# Autodesk Inventor assembly: ASY MSC 080 gills
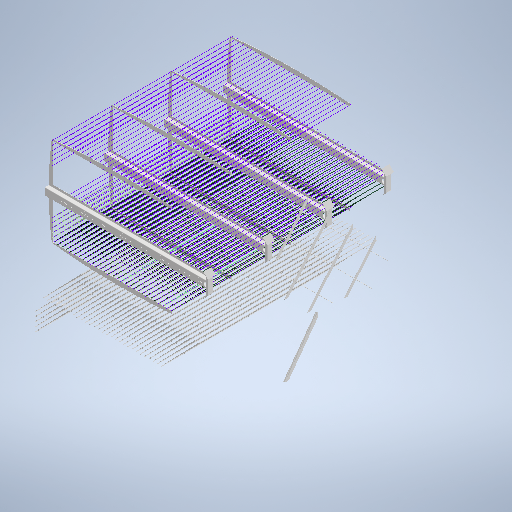
[picture p0: Inventor's stored thumbnail of the model, 512x512]
Saved by Autodesk Inventor 2025 (Build 290162010, 162A)
## iProperties
Created: 2024-08-31
Part Number: ASY MSC 080 gills
Document SubType Name: Assembly
Designer: pokla
Stock Number: ASY МОО 080 Жабры
Author: pokla
## Documents named in this file (25)
- C:\Users\DELL\YandexDisk-badmisterfox\домашниий пк\Inventor\Manturovo\Manturovo_Se-clar\ASY MSC 080 gills.iam
- C:\Users\DELL\YandexDisk-badmisterfox\домашниий пк\Inventor\Manturovo\Manturovo_Se-clar\MSC 802 sheet gills.ipt
- C:\Users\DELL\YandexDisk-badmisterfox\домашниий пк\Inventor\Manturovo\Manturovo_Se-clar\MSC 081 pillar gills.ipt
- C:\Users\DELL\YandexDisk-badmisterfox\домашниий пк\Inventor\Manturovo\Manturovo_Se-clar\MSC 804 sheet gills.ipt
- C:\Users\DELL\YandexDisk-badmisterfox\домашниий пк\Inventor\Manturovo\Manturovo_Se-clar\MSC 803 sheet gills.ipt
- C:\Users\DELL\YandexDisk-badmisterfox\домашниий пк\Inventor\Manturovo\Manturovo_Se-clar\MSC 806 sheet gills.ipt
- C:\Users\DELL\YandexDisk-badmisterfox\домашниий пк\Inventor\Manturovo\Manturovo_Se-clar\MSC 805 sheet gills.ipt
- C:\Users\DELL\YandexDisk-badmisterfox\домашниий пк\Inventor\Manturovo\Manturovo_Se-clar\MSC 808 sheet gills.ipt
- C:\Users\DELL\YandexDisk-badmisterfox\домашниий пк\Inventor\Manturovo\Manturovo_Se-clar\MSC 807 sheet gills.ipt
- C:\Users\DELL\YandexDisk-badmisterfox\домашниий пк\Inventor\Manturovo\Manturovo_Se-clar\MSC 810 sheet gills.ipt
- C:\Users\DELL\YandexDisk-badmisterfox\домашниий пк\Inventor\Manturovo\Manturovo_Se-clar\MSC 809 sheet gills.ipt
- C:\Users\DELL\YandexDisk-badmisterfox\домашниий пк\Inventor\Manturovo\Manturovo_Se-clar\MSC 812 sheet gills.ipt
- C:\Users\DELL\YandexDisk-badmisterfox\домашниий пк\Inventor\Manturovo\Manturovo_Se-clar\MSC 811 sheet gills.ipt
- C:\Users\DELL\YandexDisk-badmisterfox\домашниий пк\Inventor\Manturovo\Manturovo_Se-clar\MSC 084 wall support gills.ipt
- C:\Users\DELL\YandexDisk-badmisterfox\домашниий пк\Inventor\Manturovo\Manturovo_Se-clar\MSC 082 pillar gills.ipt
- C:\Users\DELL\YandexDisk-badmisterfox\домашниий пк\Inventor\Manturovo\Manturovo_Se-clar\MSC 086 string for sheets gills.ipt
- C:\Users\DELL\YandexDisk-badmisterfox\домашниий пк\Inventor\Manturovo\Manturovo_Se-clar\MSC 083 top support gills.ipt
- C:\Users\DELL\YandexDisk-badmisterfox\домашниий пк\Inventor\Manturovo\Manturovo_Se-clar\MSC 801 sheet gills.ipt
- C:\Users\DELL\YandexDisk-badmisterfox\домашниий пк\Inventor\Manturovo\Manturovo_Se-clar\ASY MSC 089 gills base.iam
- C:\Users\DELL\YandexDisk-badmisterfox\домашниий пк\Inventor\Manturovo\Manturovo_Se-clar\MSC 082 pillar 2.ipt
- C:\Users\DELL\YandexDisk-badmisterfox\домашниий пк\Inventor\Manturovo\Manturovo_Se-clar\MSC 0691 stringer cone.ipt
- C:\Users\DELL\YandexDisk-badmisterfox\домашниий пк\Inventor\Manturovo\Manturovo_Se-clar\конус\MSC 0161 stringer cone exit back.ipt
- C:\Users\DELL\YandexDisk-badmisterfox\домашниий пк\Inventor\Manturovo\Manturovo_Se-clar\конус\MSC 0162 stringer cone exit back.ipt
- C:\Users\DELL\YandexDisk-badmisterfox\домашниий пк\Inventor\Manturovo\Manturovo_Se-clar\конус\MSC 0163 rib cone exit back.ipt
- C:\Users\DELL\YandexDisk-badmisterfox\домашниий пк\Inventor\Manturovo\Manturovo_Se-clar\конус\MSC 0164 rib cone exit back.ipt
## Components (347 placed, 35 different names)
1. MSC 804 sheet gills:1 — Rigid:39
2. MSC 803 sheet gills:1 — Angle:2, Tangent:8, Tangent:9, Flush:15, Flush:19, Rigid:39
3. MSC 806 sheet gills:1 — Rigid:36
4. MSC 805 sheet gills:1 — Rigid:36, Angle:3, Tangent:10, Tangent:11, Flush:15, Flush:16
5. MSC 808 sheet gills:1 — Rigid:37
6. MSC 807 sheet gills:1 — Rigid:37, Angle:4, Tangent:12, Tangent:13, Flush:16, Flush:17
7. MSC 810 sheet gills:1 — Rigid:38
8. MSC 809 sheet gills:1 — Rigid:38, Angle:5, Tangent:17, Tangent:18, Flush:17, Flush:18
9. MSC 812 sheet gills:1 — Rigid:32
10. MSC 811 sheet gills:1 — Rigid:32, Angle:6, Tangent:19, Tangent:20, Flush:18
11. MSC 084 wall support gills:1 — Rigid:12, Rigid:25, Rigid:30, Tangent:14, Tangent:15
12. MSC 084 wall support gills:2 — Rigid:25, Rigid:26, Mate:17
13. MSC 084 wall support gills:3 — Rigid:26, Rigid:27
14. MSC 084 wall support gills:4 — Rigid:27
15. MSC 0103 sheet gills:2
16. MSC 0203 sheet gills:2
17. MSC 0104 sheet gills:2
18. MSC 0204 sheet gills:2
19. MSC 0105 sheet gills:2
20. MSC 0205 sheet gills:2
21. MSC 0106 sheet gills:2
22. MSC 0206 sheet gills:2
23. MSC 0107 sheet gills:2
24. MSC 0207 sheet gills:2
25. MSC 0161 stringer cone exit back:1
26. MSC 0162 stringer cone exit back:1
27. MSC 0161 stringer cone exit back:2
28. MSC 0162 stringer cone exit back:2
29. MSC 0163 rib cone exit back:1
30. MSC 0164 rib cone exit back:1
31. MSC 0163 rib cone exit back:2
32. MSC 081 pillar gills:1 — Rotational:1, Rotational:2, Tangent:16, Mate:18
33. MSC 082 pillar gills:1 — Rigid:28, Rigid:29
34. ASY MSC 089 gills base:1 [sub-assembly]
35. MSC 083 top support gills:1 — Rigid:24, Rigid:29, Rigid:31
36. MSC 083 top support gills:2 — Rigid:28, Rigid:30, Tangent:8, Tangent:9, Tangent:10, Tangent:11, Tangent:12, Tangent:13, Tangent:17, Tangent:18, Tangent:19, Tangent:20, Rigid:40
37. MSC 084 wall support gills:5 — Rigid:15, Rigid:31
38. MSC 081 pillar gills:2
39. MSC 082 pillar gills:2
40. ASY MSC 089 gills base:2 [sub-assembly]
41. MSC 083 top support gills:3
42. MSC 083 top support gills:6
43. MSC 084 wall support gills:6
44. MSC 081 pillar gills:3
45. MSC 082 pillar gills:3
46. ASY MSC 089 gills base:3 [sub-assembly]
47. MSC 083 top support gills:4
48. MSC 083 top support gills:7
49. MSC 084 wall support gills:7
50. MSC 081 pillar gills:4
51. MSC 082 pillar gills:4
52. ASY MSC 089 gills base:4 [sub-assembly]
53. MSC 083 top support gills:5
54. MSC 083 top support gills:8
55. MSC 084 wall support gills:8
56. MSC 801 sheet gills:1 — Mate:17, Rigid:33, Angle:2, Angle:3, Angle:4, Angle:5, Angle:6, Tangent:14, Tangent:15, Tangent:16, Flush:19
57. MSC 802 sheet gills:1 — Rigid:33
58. MSC 802 sheet gills:2
59. MSC 0201 sheet gills:2
60. MSC 0201 sheet gills:3
61. MSC 802 sheet gills:3
62. MSC 802 sheet gills:4
63. MSC 0201 sheet gills:4
64. MSC 0201 sheet gills:5
65. MSC 802 sheet gills:5
66. MSC 802 sheet gills:6
67. MSC 0201 sheet gills:6
68. MSC 0201 sheet gills:7
69. MSC 802 sheet gills:7
70. MSC 802 sheet gills:8
71. MSC 0201 sheet gills:8
72. MSC 0201 sheet gills:9
73. MSC 802 sheet gills:9
74. MSC 802 sheet gills:10
75. MSC 0201 sheet gills:10
76. MSC 0201 sheet gills:11
77. MSC 802 sheet gills:11
78. MSC 802 sheet gills:12
79. MSC 0201 sheet gills:12
80. MSC 0201 sheet gills:13
81. MSC 802 sheet gills:13
82. MSC 802 sheet gills:14
83. MSC 0201 sheet gills:14
84. MSC 0201 sheet gills:15
85. MSC 802 sheet gills:15
86. MSC 802 sheet gills:16
87. MSC 0201 sheet gills:16
88. MSC 0201 sheet gills:17
89. MSC 802 sheet gills:17
90. MSC 802 sheet gills:18
91. MSC 0201 sheet gills:18
92. MSC 0201 sheet gills:19
93. MSC 802 sheet gills:19
94. MSC 802 sheet gills:20
95. MSC 0201 sheet gills:20
96. MSC 0201 sheet gills:21
97. MSC 802 sheet gills:21
98. MSC 802 sheet gills:22
99. MSC 0201 sheet gills:22
100. MSC 0201 sheet gills:23
101. MSC 802 sheet gills:23
102. MSC 802 sheet gills:24
103. MSC 0201 sheet gills:24
104. MSC 0201 sheet gills:25
105. MSC 802 sheet gills:25
106. MSC 802 sheet gills:26
107. MSC 0201 sheet gills:26
108. MSC 0201 sheet gills:27
109. MSC 802 sheet gills:27
110. MSC 802 sheet gills:28
111. MSC 0201 sheet gills:28
112. MSC 0201 sheet gills:29
113. MSC 802 sheet gills:29
114. MSC 802 sheet gills:30
115. MSC 0201 sheet gills:30
116. MSC 0201 sheet gills:31
117. MSC 802 sheet gills:31
118. MSC 802 sheet gills:32
119. MSC 0201 sheet gills:32
120. MSC 0201 sheet gills:33
121. MSC 802 sheet gills:33
122. MSC 802 sheet gills:34
123. MSC 0201 sheet gills:34
124. MSC 0201 sheet gills:35
125. MSC 802 sheet gills:35
126. MSC 802 sheet gills:36
127. MSC 0201 sheet gills:36
128. MSC 0201 sheet gills:37
129. MSC 802 sheet gills:37
130. MSC 802 sheet gills:38
131. MSC 0201 sheet gills:38
132. MSC 0201 sheet gills:39
133. MSC 802 sheet gills:39
134. MSC 802 sheet gills:40
135. MSC 0201 sheet gills:40
136. MSC 0201 sheet gills:41
137. MSC 802 sheet gills:41
138. MSC 802 sheet gills:42
139. MSC 0201 sheet gills:42
140. MSC 0201 sheet gills:43
141. MSC 802 sheet gills:43
142. MSC 802 sheet gills:44
143. MSC 0201 sheet gills:44
144. MSC 0201 sheet gills:45
145. MSC 802 sheet gills:45
146. MSC 802 sheet gills:46
147. MSC 0201 sheet gills:46
148. MSC 0201 sheet gills:47
149. MSC 802 sheet gills:47
150. MSC 802 sheet gills:48
151. MSC 0201 sheet gills:48
152. MSC 0201 sheet gills:49
153. MSC 802 sheet gills:49
154. MSC 802 sheet gills:50
155. MSC 0201 sheet gills:50
156. MSC 0201 sheet gills:51
157. MSC 802 sheet gills:51
158. MSC 802 sheet gills:52
159. MSC 0201 sheet gills:52
160. MSC 0201 sheet gills:53
161. MSC 802 sheet gills:53
162. MSC 802 sheet gills:54
163. MSC 0201 sheet gills:54
164. MSC 0201 sheet gills:55
165. MSC 802 sheet gills:55
166. MSC 802 sheet gills:56
167. MSC 0201 sheet gills:56
168. MSC 0201 sheet gills:57
169. MSC 802 sheet gills:57
170. MSC 802 sheet gills:58
171. MSC 0201 sheet gills:58
172. MSC 086 string for sheets gills:1 — Rigid:12
173. MSC 086 string for sheets gills:2 — Rigid:15
174. MSC 086 string for sheets gills:3
175. MSC 086 string for sheets gills:344
176. MSC 086 string for sheets gills:5
177. MSC 086 string for sheets gills:345
178. MSC 086 string for sheets gills:7
179. MSC 086 string for sheets gills:346
180. MSC 086 string for sheets gills:9
181. MSC 086 string for sheets gills:347
182. MSC 086 string for sheets gills:11
183. MSC 086 string for sheets gills:348
184. MSC 086 string for sheets gills:13
185. MSC 086 string for sheets gills:349
186. MSC 086 string for sheets gills:15
187. MSC 086 string for sheets gills:350
188. MSC 086 string for sheets gills:17
189. MSC 086 string for sheets gills:351
190. MSC 086 string for sheets gills:19
191. MSC 086 string for sheets gills:352
192. MSC 086 string for sheets gills:21
193. MSC 086 string for sheets gills:353
194. MSC 086 string for sheets gills:23
195. MSC 086 string for sheets gills:354
196. MSC 086 string for sheets gills:25
197. MSC 086 string for sheets gills:355
198. MSC 086 string for sheets gills:27
199. MSC 086 string for sheets gills:356
200. MSC 086 string for sheets gills:29
201. MSC 086 string for sheets gills:357
202. MSC 086 string for sheets gills:31
203. MSC 086 string for sheets gills:358
204. MSC 086 string for sheets gills:33
205. MSC 086 string for sheets gills:359
206. MSC 086 string for sheets gills:35
207. MSC 086 string for sheets gills:360
208. MSC 086 string for sheets gills:37
209. MSC 086 string for sheets gills:361
210. MSC 086 string for sheets gills:39
211. MSC 086 string for sheets gills:362
212. MSC 086 string for sheets gills:41
213. MSC 086 string for sheets gills:363
214. MSC 086 string for sheets gills:43
215. MSC 086 string for sheets gills:364
216. MSC 086 string for sheets gills:45
217. MSC 086 string for sheets gills:365
218. MSC 086 string for sheets gills:47
219. MSC 086 string for sheets gills:366
220. MSC 086 string for sheets gills:49
221. MSC 086 string for sheets gills:367
222. MSC 086 string for sheets gills:51
223. MSC 086 string for sheets gills:368
224. MSC 086 string for sheets gills:53
225. MSC 086 string for sheets gills:369
226. MSC 086 string for sheets gills:55
227. MSC 086 string for sheets gills:370
228. MSC 086 string for sheets gills:58 — Rotational:1
229. MSC 086 string for sheets gills:57 — Rotational:2
230. MSC 082 pillar 2:1 — Mate:18
231. MSC 086 string for sheets gills:278
232. MSC 086 string for sheets gills:279
233. MSC 082 pillar 2:2
234. MSC 086 string for sheets gills:280
235. MSC 086 string for sheets gills:281
236. MSC 082 pillar 2:3
237. MSC 086 string for sheets gills:282
238. MSC 086 string for sheets gills:283
239. MSC 082 pillar 2:4
240. MSC 086 string for sheets gills:284
241. MSC 086 string for sheets gills:285
242. MSC 082 pillar 2:5
243. MSC 086 string for sheets gills:286
244. MSC 086 string for sheets gills:287
245. MSC 082 pillar 2:6
246. MSC 086 string for sheets gills:288
247. MSC 086 string for sheets gills:289
248. MSC 082 pillar 2:7
249. MSC 086 string for sheets gills:290
250. MSC 086 string for sheets gills:291
251. MSC 082 pillar 2:8
252. MSC 086 string for sheets gills:292
253. MSC 086 string for sheets gills:293
254. MSC 082 pillar 2:9
255. MSC 086 string for sheets gills:294
256. MSC 086 string for sheets gills:295
257. MSC 082 pillar 2:10
258. MSC 086 string for sheets gills:296
259. MSC 086 string for sheets gills:297
260. MSC 082 pillar 2:11
261. MSC 086 string for sheets gills:298
262. MSC 086 string for sheets gills:299
263. MSC 082 pillar 2:12
264. MSC 086 string for sheets gills:300
265. MSC 086 string for sheets gills:301
266. MSC 082 pillar 2:13
267. MSC 086 string for sheets gills:302
268. MSC 086 string for sheets gills:303
269. MSC 082 pillar 2:14
270. MSC 086 string for sheets gills:304
271. MSC 086 string for sheets gills:305
272. MSC 082 pillar 2:15
273. MSC 086 string for sheets gills:306
274. MSC 086 string for sheets gills:307
275. MSC 082 pillar 2:16
276. MSC 086 string for sheets gills:308
277. MSC 086 string for sheets gills:309
278. MSC 082 pillar 2:17
279. MSC 086 string for sheets gills:310
280. MSC 086 string for sheets gills:311
281. MSC 082 pillar 2:18
282. MSC 086 string for sheets gills:312
283. MSC 086 string for sheets gills:313
284. MSC 082 pillar 2:19
285. MSC 086 string for sheets gills:314
286. MSC 086 string for sheets gills:315
287. MSC 082 pillar 2:20
288. MSC 086 string for sheets gills:316
289. MSC 086 string for sheets gills:317
290. MSC 082 pillar 2:21
291. MSC 086 string for sheets gills:318
292. MSC 086 string for sheets gills:319
293. MSC 082 pillar 2:22
294. MSC 086 string for sheets gills:320
295. MSC 086 string for sheets gills:321
296. MSC 082 pillar 2:23
297. MSC 086 string for sheets gills:322
298. MSC 086 string for sheets gills:323
299. MSC 082 pillar 2:24
300. MSC 086 string for sheets gills:324
301. MSC 086 string for sheets gills:325
302. MSC 082 pillar 2:25
303. MSC 086 string for sheets gills:326
304. MSC 086 string for sheets gills:327
305. MSC 082 pillar 2:26
306. MSC 086 string for sheets gills:328
307. MSC 086 string for sheets gills:329
308. MSC 082 pillar 2:27
309. MSC 086 string for sheets gills:330
310. MSC 086 string for sheets gills:331
311. MSC 082 pillar 2:28
312. MSC 086 string for sheets gills:332
313. MSC 086 string for sheets gills:333
314. MSC 082 pillar 2:29
315. MSC 086 string for sheets gills:334
316. MSC 086 string for sheets gills:335
317. MSC 082 pillar 2:30
318. MSC 086 string for sheets gills:336
319. MSC 086 string for sheets gills:337
320. MSC 082 pillar 2:31
321. MSC 086 string for sheets gills:338
322. MSC 086 string for sheets gills:339
323. MSC 082 pillar 2:32
324. MSC 086 string for sheets gills:340
325. MSC 086 string for sheets gills:341
326. MSC 082 pillar 2:33
327. MSC 086 string for sheets gills:342
328. MSC 086 string for sheets gills:343
329. MSC 082 pillar 2:34
330. MSC 086 string for sheets gills:125 — Rigid:40
331. MSC 086 string for sheets gills:126
332. MSC 086 string for sheets gills:127
333. MSC 086 string for sheets gills:128
334. MSC 086 string for sheets gills:129
335. MSC 086 string for sheets gills:130
336. MSC 086 string for sheets gills:131 — Rigid:24
337. MSC 086 string for sheets gills:371
338. MSC 086 string for sheets gills:372
339. MSC 086 string for sheets gills:373
340. MSC 086 string for sheets gills:374
341. MSC 086 string for sheets gills:375
342. MSC 0691 stringer cone:1
343. MSC 0691 stringer cone:2
344. MSC 0691 stringer cone:3
345. MSC 0691 stringer cone:4
346. MSC 0691 stringer cone:5
347. MSC 0691 stringer cone:6
## Component patterns: (4 elements, first: MSC 081 pillar gills:1 + MSC 082 pillar gills:1 + ASY MSC 089 gills base:1 + MSC 083 top support gills:1 + MSC 083 top support gills:2 + MSC 084 wall support gills:5), (29 elements, first: MSC 801 sheet gills:1 + MSC 802 sheet gills:1 + MSC 802 sheet gills:2 + MSC 0201 sheet gills:2), (28 elements, first: MSC 086 string for sheets gills:1 + MSC 086 string for sheets gills:2), (34 elements, first: MSC 086 string for sheets gills:58 + MSC 086 string for sheets gills:57 + MSC 082 pillar 2:1), (6 elements, first: MSC 086 string for sheets gills:125), (6 elements, first: MSC 086 string for sheets gills:131), (6 elements, first: MSC 0691 stringer cone:1)
## Relationships (67: WeldJoint 30, Tangent 13, Flush 12, Mate 5, Angle 5, RevoluteJoint 2)
- [WeldJoint]: MSC 081 pillar gills:1 ↔ MSC 082 pillar gills:1
- [Flush]: MSC 081 pillar gills:1 ↔ ASY MSC 089 gills base:1
- [Mate]: MSC 081 pillar gills:1 ↔ ASY MSC 089 gills base:1
- [Flush] (5 mm): MSC 081 pillar gills:1 ↔ ASY MSC 089 gills base:1
- Rigid:12 [WeldJoint] (-5 mm): MSC 084 wall support gills:1 ↔ MSC 086 string for sheets gills:1
- Rigid:15 [WeldJoint] (-5 mm): MSC 084 wall support gills:5 ↔ MSC 086 string for sheets gills:2
- [Mate]: ASY MSC 089 gills base:1
- [Mate]: ASY MSC 089 gills base:1
- [Flush]: ASY MSC 089 gills base:1
- Rigid:24 [WeldJoint] (-5 mm): MSC 083 top support gills:1 ↔ MSC 086 string for sheets gills:131
- Rigid:25 [WeldJoint] (985 mm): MSC 084 wall support gills:1 ↔ MSC 084 wall support gills:2
- Rigid:26 [WeldJoint] (985 mm): MSC 084 wall support gills:2 ↔ MSC 084 wall support gills:3
- Rigid:27 [WeldJoint] (985 mm): MSC 084 wall support gills:3 ↔ MSC 084 wall support gills:4
- Mate:17: MSC 084 wall support gills:2 ↔ MSC 801 sheet gills:1
- Rigid:28 [WeldJoint]: MSC 082 pillar gills:1 ↔ MSC 083 top support gills:2
- Rigid:29 [WeldJoint]: MSC 082 pillar gills:1 ↔ MSC 083 top support gills:1
- Rigid:30 [WeldJoint]: MSC 084 wall support gills:1 ↔ MSC 083 top support gills:2
- Rigid:31 [WeldJoint]: MSC 083 top support gills:1 ↔ MSC 084 wall support gills:5
- Rotational:1 [RevoluteJoint] (5 mm): MSC 081 pillar gills:1 ↔ MSC 086 string for sheets gills:58
- Rotational:2 [RevoluteJoint] (-5 mm): MSC 081 pillar gills:1 ↔ MSC 086 string for sheets gills:57
- Rigid:32 [WeldJoint] (-10 mm): MSC 812 sheet gills:1 ↔ MSC 811 sheet gills:1
- Rigid:33 [WeldJoint] (-10 mm): MSC 801 sheet gills:1 ↔ MSC 802 sheet gills:1
- Rigid:36 [WeldJoint] (-10 mm): MSC 806 sheet gills:1 ↔ MSC 805 sheet gills:1
- Rigid:37 [WeldJoint] (-10 mm): MSC 808 sheet gills:1 ↔ MSC 807 sheet gills:1
- Rigid:38 [WeldJoint] (-10 mm): MSC 810 sheet gills:1 ↔ MSC 809 sheet gills:1
- Angle:2 (0 deg): MSC 803 sheet gills:1 ↔ MSC 801 sheet gills:1
- Angle:3 (0 deg): MSC 805 sheet gills:1 ↔ MSC 801 sheet gills:1
- Angle:4 (0 deg): MSC 807 sheet gills:1 ↔ MSC 801 sheet gills:1
- Angle:5 (0 deg): MSC 809 sheet gills:1 ↔ MSC 801 sheet gills:1
- Angle:6 (0 deg): MSC 811 sheet gills:1 ↔ MSC 801 sheet gills:1
- Tangent:8: MSC 803 sheet gills:1 ↔ MSC 083 top support gills:2
- Tangent:9: MSC 803 sheet gills:1 ↔ MSC 083 top support gills:2
- Tangent:10: MSC 805 sheet gills:1 ↔ MSC 083 top support gills:2
- Tangent:11: MSC 805 sheet gills:1 ↔ MSC 083 top support gills:2
- Tangent:12: MSC 807 sheet gills:1 ↔ MSC 083 top support gills:2
- Tangent:13: MSC 807 sheet gills:1 ↔ MSC 083 top support gills:2
- Tangent:14: MSC 084 wall support gills:1 ↔ MSC 801 sheet gills:1
- Tangent:15: MSC 084 wall support gills:1 ↔ MSC 801 sheet gills:1
- Tangent:16: MSC 081 pillar gills:1 ↔ MSC 801 sheet gills:1
- Tangent:17: MSC 809 sheet gills:1 ↔ MSC 083 top support gills:2
- Tangent:18: MSC 809 sheet gills:1 ↔ MSC 083 top support gills:2
- Tangent:19: MSC 811 sheet gills:1 ↔ MSC 083 top support gills:2
- Tangent:20: MSC 811 sheet gills:1 ↔ MSC 083 top support gills:2
- Flush:15: MSC 803 sheet gills:1 ↔ MSC 805 sheet gills:1
- Flush:16: MSC 805 sheet gills:1 ↔ MSC 807 sheet gills:1
- Flush:17: MSC 807 sheet gills:1 ↔ MSC 809 sheet gills:1
- Flush:18: MSC 809 sheet gills:1 ↔ MSC 811 sheet gills:1
- Flush:19: MSC 803 sheet gills:1 ↔ MSC 801 sheet gills:1
- Rigid:39 [WeldJoint] (-10 mm): MSC 804 sheet gills:1 ↔ MSC 803 sheet gills:1
- Rigid:40 [WeldJoint] (5 mm): MSC 083 top support gills:2 ↔ MSC 086 string for sheets gills:125
- [WeldJoint] (-10 mm): MSC 802 sheet gills:2 ↔ MSC 0201 sheet gills:2
- [WeldJoint] (-10 mm): MSC 0107 sheet gills:2 ↔ MSC 0207 sheet gills:2
- [WeldJoint] (-10 mm): MSC 0104 sheet gills:2 ↔ MSC 0204 sheet gills:2
- [WeldJoint] (-10 mm): MSC 0105 sheet gills:2 ↔ MSC 0205 sheet gills:2
- [WeldJoint] (-10 mm): MSC 0106 sheet gills:2 ↔ MSC 0206 sheet gills:2
- [Flush]: MSC 0203 sheet gills:2 ↔ MSC 0204 sheet gills:2
- [Flush]: MSC 0204 sheet gills:2 ↔ MSC 0205 sheet gills:2
- [Flush]: MSC 0205 sheet gills:2 ↔ MSC 0206 sheet gills:2
- [Flush]: MSC 0206 sheet gills:2 ↔ MSC 0207 sheet gills:2
- [WeldJoint] (-10 mm): MSC 0103 sheet gills:2 ↔ MSC 0203 sheet gills:2
- Mate:18: MSC 081 pillar gills:1 ↔ MSC 082 pillar 2:1
- [WeldJoint] (374 mm): MSC 0163 rib cone exit back:1 ↔ MSC 0163 rib cone exit back:2
- [WeldJoint] (374 mm): MSC 0164 rib cone exit back:1 ↔ MSC 0163 rib cone exit back:2
- [WeldJoint] (2 mm): MSC 0162 stringer cone exit back:1 ↔ MSC 0163 rib cone exit back:1
- [WeldJoint] (2 mm): MSC 0162 stringer cone exit back:2 ↔ MSC 0163 rib cone exit back:1
- [WeldJoint] (2 mm): MSC 0161 stringer cone exit back:1 ↔ MSC 0163 rib cone exit back:1
- [WeldJoint] (2 mm): MSC 0161 stringer cone exit back:2 ↔ MSC 0163 rib cone exit back:1
## Named parameters: d233_d176 = -10 mm, d234_d202 = 0 mm, d235_d203 = 0 mm, d236_d204 = 0 mm, d237_d205 = 0 mm, d238_d207 = -10 mm, d239_d180 = -10 mm, d240_d181 = -10 mm, d241_d173 = -10 mm, d242_d179 = -10 mm
